# Autodesk Inventor assembly: SolarPanel
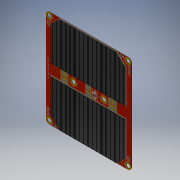
[picture p0: Inventor's stored thumbnail of the model, 180x180]
Saved by Autodesk Inventor 2018 (Build 220112000, 112)
## iProperties
Created: 2018-11-29
Part Number: SolarPanel
Document SubType Name: Assembly
Designer: Bradley
Author: Bradley
## Documents named in this file (8)
- C:\Users\Bradley\Documents\GitHub\CougSat1-Hardware\CougSat1-PowerBoard\CADModel\Native\SolarPanel.iam
- C:\Users\Bradley\Documents\GitHub\CougSat1-Hardware\CougSat1-PowerBoard\CADModel\Native\SolarPanel_PCB.ipt
- C:\Users\Bradley\Documents\GitHub\Resources\SupplierDocuments\04 - Connectors SMT\04-0001\04-0001.iam
- C:\Users\Bradley\Documents\GitHub\Resources\SupplierDocuments\04 - Connectors SMT\04-0007\04-0007.iam
- C:\Users\Bradley\Documents\GitHub\Resources\SupplierDocuments\26 - Resistor Misc\26-0008\26-0008.ipt
- C:\Users\Bradley\Documents\GitHub\Resources\SupplierDocuments\02 - Solar Cell\02-0001\02-0001.ipt
- C:\Users\Bradley\Documents\GitHub\Resources\SupplierDocuments\34 - Inductor 3225 and larger\34-103A\34-103A.ipt
- C:\Users\Bradley\Documents\GitHub\Resources\SupplierDocuments\66 - Sensor\66-0003\66-0003.ipt
## Components (13 placed, 7 different names)
1. 02-0001:1 — Mate:1, Mate:3, Mate:4
2. 02-0001:2 — Mate:2, Flush:1, Flush:2
3. 04-0001:1 [sub-assembly] — Mate:49, Flush:17, Flush:18
4. 04-0007:1 [sub-assembly] — Mate:48, Flush:19, Flush:20
5. 26-0008:1 — Mate:6, Mate:7, Flush:3
6. 26-0008:2 — Mate:5, Mate:8, Flush:4
7. 26-0008:3 — Mate:58, Mate:61, Mate:62
8. 26-0008:4 — Mate:59, Mate:63, Mate:64
9. 26-0008:5 — Mate:60, Mate:65, Mate:66
10. 34-103A:1 — Mate:50, Mate:52, Flush:21
11. 34-103A:2 — Mate:51, Mate:53, Flush:22
12. 66-0003:1 — Mate:29, Mate:30, Flush:9
13. SolarPanel_PCB:1 — Mate:1, Mate:2, Mate:5, Mate:6, Mate:29, Mate:48, Mate:49, Mate:50, Mate:51, Mate:58, Mate:59, Mate:60
## Relationships (36: Mate 25, Flush 11)
- Mate:1: 02-0001:1 ↔ SolarPanel_PCB:1
- Mate:2: 02-0001:2 ↔ SolarPanel_PCB:1
- Mate:3: 02-0001:1
- Flush:1: 02-0001:2
- Flush:2 (5 mm): 02-0001:2
- Mate:4 (5 mm): 02-0001:1
- Mate:5: 26-0008:2 ↔ SolarPanel_PCB:1
- Mate:6: 26-0008:1 ↔ SolarPanel_PCB:1
- Mate:7 (31 mm): 26-0008:1
- Flush:3 (-43.5 mm): 26-0008:1
- Mate:8 (-31.125 mm): 26-0008:2
- Flush:4 (43.8 mm): 26-0008:2
- Mate:29: 66-0003:1 ↔ SolarPanel_PCB:1
- Mate:30 (-0.25 mm): 66-0003:1
- Flush:9 (-6.25 mm): 66-0003:1
- Mate:48: 04-0007:1 ↔ SolarPanel_PCB:1
- Mate:49: 04-0001:1 ↔ SolarPanel_PCB:1
- Flush:17 (26 mm): 04-0001:1
- Flush:18 (-1 mm): 04-0001:1
- Flush:19 (11.75 mm): 04-0007:1
- Flush:20 (-1 mm): 04-0007:1
- Mate:50: 34-103A:1 ↔ SolarPanel_PCB:1
- Mate:51: 34-103A:2 ↔ SolarPanel_PCB:1
- Mate:52 (-16.25 mm): 34-103A:1
- Flush:21 (8 mm): 34-103A:1
- Mate:53 (16.25 mm): 34-103A:2
- Flush:22 (-8 mm): 34-103A:2
- Mate:58: 26-0008:3 ↔ SolarPanel_PCB:1
- Mate:59: 26-0008:4 ↔ SolarPanel_PCB:1
- Mate:60: 26-0008:5 ↔ SolarPanel_PCB:1
- Mate:61 (-10.75 mm): 26-0008:3
- Mate:62 (-4.75 mm): 26-0008:3
- Mate:63 (1.85 mm): 26-0008:4
- Mate:64 (-2.6 mm): 26-0008:4
- Mate:65 (10.75 mm): 26-0008:5
- Mate:66 (4.75 mm): 26-0008:5
